# Autodesk Inventor assembly: MX-106T+idle.ipt
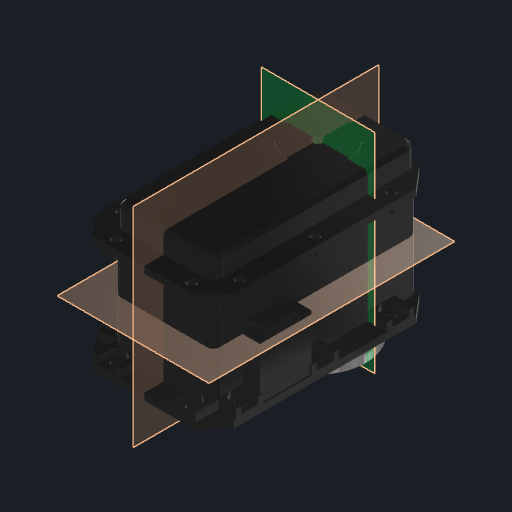
[picture p0: Inventor's stored thumbnail of the model, 512x512]
Saved by Autodesk Inventor 2024.3 (Build 283343000, 343)
## iProperties
Created: 2022-08-09
Part Number: MX-106T+idle.ipt
Document SubType Name: Assembly
Designer: 박지훈
Author: 박지훈
## Documents named in this file (3)
- C:\Users\ASUS\Desktop\Anti_Backlash_Structure_OP\ROBOTIS(Inventor 2024 ver.)\DXL\MX-106T+idle.ipt.iam
- C:\Users\ASUS\Desktop\ABD_2024_Eindhoven\ROBOTIS(Inventor 2024 ver.)\IDLER\64idler.iam
- C:\Users\ASUS\Desktop\Anti_Backlash_Structure_OP\ROBOTIS(Inventor 2024 ver.)\DXL\MX-106T.ipt
## Components (2 placed, 2 different names)
1. 64idler:1 [sub-assembly] — 삽입:1
2. MX-106T:1 — 삽입:1
## Relationships (1: Insert 1)
- 삽입:1 [Insert] (0.06 mm): 64idler:1 ↔ MX-106T:1
